# Autodesk Inventor assembly: mag_6mm
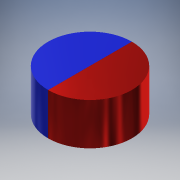
[picture p0: Inventor's stored thumbnail of the model, 180x180]
Saved by Autodesk Inventor 2017 (Build 210142000, 142)
## iProperties
Created: 2020-11-15
Part Number: mag_6mm
Document SubType Name: Assembly
Designer: paulg
Author: paulg
## Documents named in this file (2)
- C:\play\3D_play\Cycloid CAD\mag_6mm.iam
- C:\play\3D_play\Cycloid CAD\half_mag.ipt
## Components (2 placed, 1 different names)
1. half_mag:1 — Mate:1, Flush:1, Insert:1
2. half_mag:2 — Mate:1, Flush:1, Insert:1
## Relationships (3: Mate 1, Flush 1, Insert 1)
- Mate:1: half_mag:1 ↔ half_mag:2
- Flush:1: half_mag:1 ↔ half_mag:2
- Insert:1: half_mag:1 ↔ half_mag:2
